# Autodesk Inventor assembly: cable-carrier
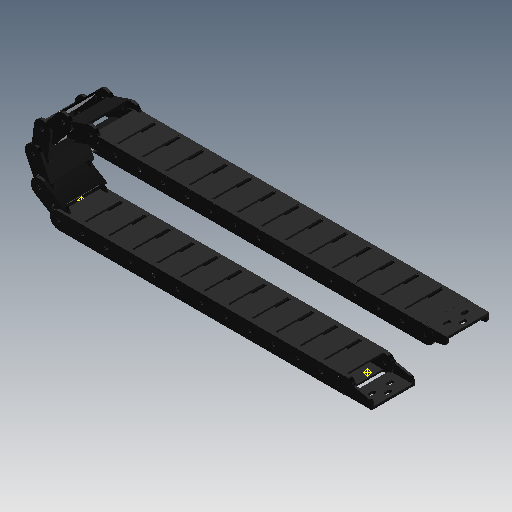
[picture p0: Inventor's stored thumbnail of the model, 512x512]
Saved by Autodesk Inventor 2017 (Build 210142000, 142)
## iProperties
Created: 2018-06-20
Part Number: cable-carrier
Document SubType Name: Assembly
Designer: Luiz Gustavo
Author: Luiz Gustavo
## Documents named in this file (4)
- C:\Users\Luiz Gustavo\Documents\Inventor\piano-robot\cable-carrier.iam
- C:\Users\Luiz Gustavo\Documents\Inventor\piano-robot\carrier-end.ipt
- C:\Users\Luiz Gustavo\Documents\Inventor\piano-robot\carrier-path.ipt
- C:\Users\Luiz Gustavo\Documents\Inventor\piano-robot\carrier-link.ipt
## Components (34 placed, 3 different names)
1. carrier-end:1 — Flush:1, Flush:2, Flush:3, Rigid:1
2. carrier-path:1 — Flush:6
3. carrier-end:2 — Flush:7, Mate:1, Flush:8
4. carrier-link:1 — Rigid:1
5. carrier-link:2
6. carrier-link:3
7. carrier-link:4
8. carrier-link:5
9. carrier-link:6
10. carrier-link:7
11. carrier-link:8
12. carrier-link:9
13. carrier-link:10
14. carrier-link:11
15. carrier-link:12
16. carrier-link:13
17. carrier-link:14
18. carrier-link:15
19. carrier-link:16
20. carrier-link:17
21. carrier-link:18
22. carrier-link:19
23. carrier-link:20
24. carrier-link:21
25. carrier-link:22
26. carrier-link:23
27. carrier-link:24
28. carrier-link:25
29. carrier-link:26
30. carrier-link:27
31. carrier-link:28
32. carrier-link:29
33. carrier-link:30
34. carrier-link:31
## Component patterns: (31 elements, first: carrier-link:1)
## Relationships (8: Flush 6, WeldJoint 1, Mate 1)
- Flush:1: carrier-end:1
- Flush:2: carrier-end:1
- Flush:3: carrier-end:1
- Flush:6: carrier-path:1
- Rigid:1 [WeldJoint]: carrier-end:1 ↔ carrier-link:1
- Flush:7 (-130 mm): carrier-end:2
- Mate:1: carrier-end:2
- Flush:8 (-105 mm): carrier-end:2
